# Autodesk Inventor assembly: Transmissão de correias sincronizadas
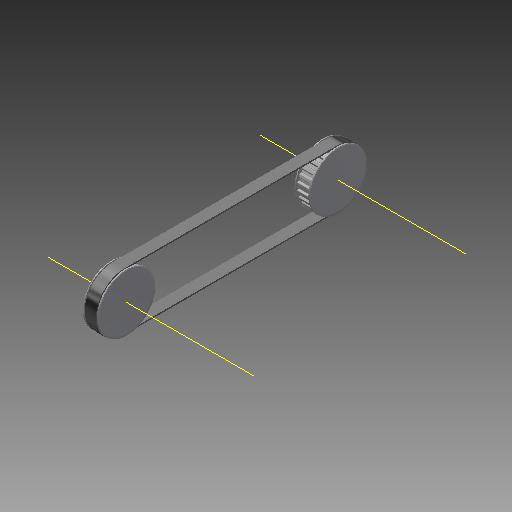
[picture p0: Inventor's stored thumbnail of the model, 512x512]
Saved by Autodesk Inventor 2018 (Build 220112000, 112)
## iProperties
ClientObjectVersion: 1
Created: 2018-09-22
Part Number: Transmissão de correias sincronizadas
Document SubType Name: Assembly
Designer: Usuario
Author: Usuario
## Documents named in this file (4)
- C:\Users\Usuario\Desktop\Estação BGA\Peças 3D\estação_bga_3\Design Accelerator\Transmissão de correias sincronizadas1.iam
- C:\Users\Usuario\Desktop\Estação BGA\Peças 3D\estação_bga_3\Design Accelerator\Correia síncrona1.ipt
- C:\Users\Usuario\Desktop\Estação BGA\Peças 3D\estação_bga_3\Design Accelerator\Polia síncrona11.ipt
- C:\Users\Usuario\Desktop\Estação BGA\Peças 3D\estação_bga_3\Design Accelerator\Polia síncrona21.ipt
## Components (3 placed, 3 different names)
1. Correia síncrona:1 — Alinhamento:1, Coincidência:1, Coincidência:2, Alinhamento:2, Coincidência:3, Coincidência:4
2. Polia síncrona1:1 — Alinhamento:1, Coincidência:1, Coincidência:2, Rotação:1
3. Polia síncrona2:1 — Alinhamento:2, Coincidência:3, Rotação:1, Coincidência:4
## Relationships (7: Mate 4, Flush 2, RelateRotation 1)
- Alinhamento:1 [Flush]: Correia síncrona:1 ↔ Polia síncrona1:1
- Coincidência:1 [Mate]: Correia síncrona:1 ↔ Polia síncrona1:1
- Coincidência:2 [Mate]: Correia síncrona:1 ↔ Polia síncrona1:1
- Alinhamento:2 [Flush]: Correia síncrona:1 ↔ Polia síncrona2:1
- Coincidência:3 [Mate]: Correia síncrona:1 ↔ Polia síncrona2:1
- Rotação:1 [RelateRotation] (1 ul): Polia síncrona1:1 ↔ Polia síncrona2:1
- Coincidência:4 [Mate]: Correia síncrona:1 ↔ Polia síncrona2:1
